# Autodesk Inventor assembly: Rebuild Chassis Assembly 26x28 Version with Shooter Tower
(part 2 of 2)
- Insert:77: Rebuild Shooter Tower Motor Mount Tube:1 ↔ 0.25x20 Washer:38
- Insert:78: Rebuild Shooter Tower Motor Mount Tube:1 ↔ 0.25x20 Washer:37
- Insert:79: Rebuild Snowblower Motor Mount:1 ↔ 0.25x20 Washer:39
- Insert:80: Rebuild Snowblower Motor Mount:1 ↔ 0.25x20 Washer:40
- Insert:81: Rebuild Snowblower Motor Mount:1 ↔ 0.25x20 Washer:41
- Insert:82: Rebuild Snowblower Motor Mount:1 ↔ 0.25x20 Washer:42
- Insert:83: Rebuild Shooter Tower Top Tube 1:1 ↔ 0.25x20 Washer:43
- Insert:84: Rebuild Shooter Tower Top Tube 1:1 ↔ 0.25x20 Washer:44
- Insert:85: 91257A548:1 ↔ 0.25x20 Washer:41
- Insert:86: 91257A548:2 ↔ 0.25x20 Washer:42
- Insert:87: 91257A548:3 ↔ 0.25x20 Washer:37
- Insert:88: 91257A548:4 ↔ 0.25x20 Washer:38
- Insert:89: 90630A110:22 ↔ 0.25x20 Washer:43
- Insert:90: 90630A110:21 ↔ 0.25x20 Washer:44
- Insert:91: 90630A110:24 ↔ 0.25x20 Washer:39
- Insert:92: 90630A110:23 ↔ 0.25x20 Washer:40
- Mate:324: Rebuild Shooter Tower Top Tube 1:1 ↔ Rebuild Flange Bearing Mount Tower:1
- Mate:325: Square Tube 3:1 ↔ Rebuild Flange Bearing Mount Tower Mirror:1
- Mate:326: Rebuild Shooter Tower Top Tube 1:1 ↔ Rebuild Flange Bearing Mount Tower:1
- Mate:327: Rebuild Shooter Tower Top Tube 1:1 ↔ Rebuild Flange Bearing Mount Tower:1
- Mate:328: Square Tube 3:1 ↔ Rebuild Flange Bearing Mount Tower Mirror:1
- Mate:329: Square Tube 3:1 ↔ Rebuild Flange Bearing Mount Tower Mirror:1
- Insert:93: Rebuild Gusset 4:3 ↔ 0.25x20 Washer:45
- Insert:94: Rebuild Gusset 4:3 ↔ 0.25x20 Washer:46
- Insert:95: Rebuild Gusset 4:5 ↔ 0.25x20 Washer:48
- Insert:96: Rebuild Gusset 4:5 ↔ 0.25x20 Washer:47
- Insert:97: 0.25x20 Washer:82 ↔ 91257A550:23
- Insert:98: 0.25x20 Washer:83 ↔ 91257A550:24
- Insert:99: Rebuild Flange Bearing Mount Tower Mirror:1 ↔ 91257A550:21
- Insert:100: Rebuild Flange Bearing Mount Tower Mirror:1 ↔ 91257A550:22
- Insert:101: 90630A110:26 ↔ 0.25x20 Washer:45
- Insert:102: 90630A110:25 ↔ 0.25x20 Washer:46
- Insert:103: 90630A110:27 ↔ 0.25x20 Washer:47
- Insert:104: 90630A110:28 ↔ 0.25x20 Washer:48
- Insert:105: Chassis Tower Bracket Part2:2 ↔ 0.25x20 Washer:49
- Insert:106: 0.25x20 Washer:50 ↔ Chassis Battery Mount Part1:1
- Insert:107: 0.25x20 Washer:50 ↔ 91257A548:5
- Insert:108: 0.25x20 Washer:49 ↔ 90630A110:29
- Insert:109: Chassis Tower Bracket Part2:1 ↔ 0.25x20 Washer:51
- Insert:110: 0.25x20 Washer:52 ↔ Chassis Battery Mount Part1:1
- Insert:111: 0.25x20 Washer:52 ↔ 91257A548:6
- Insert:112: 0.25x20 Washer:51 ↔ 90630A110:30
- Insert:113: Chassis Back Electronics Protector Bar:1 ↔ 0.25x20 Washer:53
- Insert:114: 0.25x20 Washer:54 ↔ Rebuild Mounting Board 3:1
- Insert:115: 0.25x20 Washer:53 ↔ 90630A110:31
- Insert:116: 0.25x20 Washer:54 ↔ 91257A548:7
- Mate:330: Chassis Part4 (26x28):1 ↔ Mounting Bracket V1.500 - (toughbox-mini - sheet metal - underside):2
- Mate:331: Chassis Part4 (26x28):1 ↔ Mounting Bracket V1.500 - (toughbox-mini - sheet metal):1
- Mate:332: Chassis Part4 (26x28):2 ↔ Mounting Bracket V1.500 - (toughbox-mini - sheet metal - underside):1
- Mate:333: Chassis Part4 (26x28):2 ↔ Mounting Bracket V1.500 - (toughbox-mini - sheet metal):2
- Mate:334: Chassis Part4 (26x28):2 ↔ Mounting Bracket V1.500 - (toughbox-mini - sheet metal):2
- Mate:335: Chassis Part4 (26x28):2 ↔ Mounting Bracket V1.500 - (toughbox-mini - sheet metal):2
- Mate:336: Chassis Part4 (26x28):1 ↔ Mounting Bracket V1.500 - (toughbox-mini - sheet metal):1
- Mate:337: Chassis Part4 (26x28):1 ↔ Mounting Bracket V1.500 - (toughbox-mini - sheet metal):1
- Mate:338: Chassis Part4 (26x28):1 ↔ Mounting Bracket V1.500 - (toughbox-mini - sheet metal - underside):2
- Mate:339: Chassis Part4 (26x28):1 ↔ Mounting Bracket V1.500 - (toughbox-mini - sheet metal - underside):2
- Mate:340: Chassis Part4 (26x28):2 ↔ Mounting Bracket V1.500 - (toughbox-mini - sheet metal - underside):1
- Mate:341: Chassis Part4 (26x28):2 ↔ Mounting Bracket V1.500 - (toughbox-mini - sheet metal - underside):1
- Insert:117: 0.25x20 Washer:56 ↔ Mounting Bracket V1.500 - (toughbox-mini - sheet metal):2
- Insert:118: 0.25x20 Washer:55 ↔ Mounting Bracket V1.500 - (toughbox-mini - sheet metal):2
- Insert:119: 0.25x20 Washer:57 ↔ Mounting Bracket V1.500 - (toughbox-mini - sheet metal):1
- Insert:120: 0.25x20 Washer:58 ↔ Mounting Bracket V1.500 - (toughbox-mini - sheet metal):1
- Insert:121: 0.25x20 Washer:60 ↔ Mounting Bracket V1.500 - (toughbox-mini - sheet metal - underside):1
- Insert:122: 0.25x20 Washer:59 ↔ Mounting Bracket V1.500 - (toughbox-mini - sheet metal - underside):1
- Insert:123: 0.25x20 Washer:61 ↔ Mounting Bracket V1.500 - (toughbox-mini - sheet metal - underside):2
- Insert:124: 0.25x20 Washer:62 ↔ Mounting Bracket V1.500 - (toughbox-mini - sheet metal - underside):2
- Insert:125: 91257A550:25 ↔ 0.25x20 Washer:56
- Insert:126: 91257A550:26 ↔ 0.25x20 Washer:55
- Insert:127: 91257A550:27 ↔ 0.25x20 Washer:57
- Insert:128: 91257A550:28 ↔ 0.25x20 Washer:58
- Insert:129: 90630A110:32 ↔ 0.25x20 Washer:60
- Insert:130: 90630A110:33 ↔ 0.25x20 Washer:59
- Insert:131: 90630A110:34 ↔ 0.25x20 Washer:62
- Insert:132: 90630A110:35 ↔ 0.25x20 Washer:61
- Mate:342: Rebuild Edge Mount 1:2 ↔ Back Brace Mount V2:1
- Flush:75: Rebuild Edge Mount 1:2 ↔ Back Brace Mount V2:1
- Mate:343 (155.2575 mm): Chassis V1.500 Part2:1 ↔ Back Brace Mount V2:1
- Mate:344: Circuit Breaker Mount:1 ↔ Back Brace Mount V2:1
- Mate:345: Circuit Breaker Mount:1 ↔ Back Brace Mount V2:1
- Mate:346: Circuit Breaker Mount:1 ↔ Back Brace Mount V2:1
- Insert:133: Rebuild Edge Mount 1:2 ↔ 0.25x20 Washer:65
- Insert:135: Rebuild Edge Mount 1:2 ↔ 0.25x20 Washer:63
- Insert:136: 0.25x20 Washer:66 ↔ Back Brace Mount V2:1
- Insert:138: 0.25x20 Washer:68 ↔ Back Brace Mount V2:1
- Insert:139: 0.25x20 Washer:69 ↔ Back Brace Mount V2:1
- Insert:140: 0.25x20 Washer:70 ↔ Back Brace Mount V2:1
- Insert:141: 0.25x20 Washer:71 ↔ Circuit Breaker Mount:1
- Insert:142: 0.25x20 Washer:72 ↔ Circuit Breaker Mount:1
- Insert:143: 91257A548:8 ↔ 0.25x20 Washer:66
- Insert:145: 91257A548:10 ↔ 0.25x20 Washer:68
- Insert:146: 90630A110:38 ↔ 0.25x20 Washer:63
- Insert:148: 90630A110:36 ↔ 0.25x20 Washer:65
- Insert:149: 92620A540:2 ↔ 0.25x20 Washer:71
- Insert:150: 92620A540:1 ↔ 0.25x20 Washer:72
- Insert:151: 90630A110:40 ↔ 0.25x20 Washer:69
- Insert:152: 90630A110:39 ↔ 0.25x20 Washer:70
- Flush:76 (0.7937 mm): Rebuild Shooter Tower Top Tube 1:1 ↔ Rebuild Snowblower Motor Mount:1
- Insert:155: Rebuild Gusset 4:4 ↔ 0.25x20 Washer:76
- Insert:156: Rebuild Gusset 4:4 ↔ 0.25x20 Washer:75
- Insert:157: 0.25x20 Washer:74 ↔ 91257A548:11
- Insert:158: 0.25x20 Washer:73 ↔ 91257A548:12
- Insert:159: 0.25x20 Washer:76 ↔ 90630A110:42
- Insert:160: 0.25x20 Washer:75 ↔ 90630A110:41
- Mate:350: Rebuild Encoder Mount 2:1 ↔ Rebuild Snowblower Motor Mount:1
- Mate:351: Rebuild Encoder Mount 2:1 ↔ Rebuild Snowblower Motor Mount:1
- Mate:352: Rebuild Encoder Mount 2:1 ↔ Rebuild Snowblower Motor Mount:1
- Insert:161: 90630A110:43 ↔ 0.25x20 Washer:79
- Insert:162: Rebuild Snowblower Motor Mount:1 ↔ 0.25x20 Washer:77
- Insert:163: 0.25x20 Washer:77 ↔ 92620A540:3
- Insert:164: Rebuild Encoder Mount 2:1 ↔ 0.25x20 Washer:78
- Insert:165: Rebuild Encoder Mount 2:1 ↔ 0.25x20 Washer:79
- Insert:166: 90630A110:44 ↔ 0.25x20 Washer:78
- Insert:167: Rebuild Snowblower Motor Mount:1 ↔ 92620A539:1
- Insert:168: Chassis V1.500 Part2:1 ↔ 0.25x20 Washer:80
- Insert:169: 0.25x20 Washer:80 ↔ 90630A110:45
- Insert:170: 0.25x20 Washer:81 ↔ Rebuild Mounting Board 3:1
- Insert:171: 0.25x20 Washer:81 ↔ 91257A548:13
- Insert:172: Rebuild Flange Bearing Mount Tower:1 ↔ 0.25x20 Washer:82
- Insert:173: Rebuild Flange Bearing Mount Tower:1 ↔ 0.25x20 Washer:83
- Insert:174: 0.25x20 Washer:84 ↔ 0.25x20 Washer:85
- Insert:175: 0.25x20 Washer:86 ↔ 0.25x20 Washer:85
- Insert:176: 0.25x20 Washer:86 ↔ 0.25x20 Washer:87
- Insert:177: 0.25x20 Washer:87 ↔ 0.25x20 Washer:88
- [Insert]: 0.25x20 Washer:89 ↔ 0.25x20 Washer:90
- [Insert]: 0.25x20 Washer:91 ↔ 0.25x20 Washer:90
- Insert:180: 0.25x20 Washer:88 ↔ 0.25x20 Washer:89
- [Insert]: 0.25x20 Washer:92 ↔ 0.25x20 Washer:93
- [Insert]: 0.25x20 Washer:94 ↔ 0.25x20 Washer:93
- [Insert]: 0.25x20 Washer:94 ↔ 0.25x20 Washer:95
- [Insert]: 0.25x20 Washer:96 ↔ 0.25x20 Washer:95
- [Insert]: 0.25x20 Washer:98 ↔ 0.25x20 Washer:97
- [Insert]: 0.25x20 Washer:99 ↔ 0.25x20 Washer:98
- [Insert]: 0.25x20 Washer:97 ↔ 0.25x20 Washer:96
- Insert:188: Rebuild Snowblower Motor Mount:1 ↔ 0.25x20 Washer:84
- Insert:189: Rebuild Snowblower Motor Mount:1 ↔ 0.25x20 Washer:92
- Angle:1 (0 deg): Rebuild Shooter Tower Motor Mount Tube:1 ↔ 92620A539:1
- Insert:190: Chassis V1.500 Part2:1 ↔ Chassis Back Electronics Protector Bar:1
- Flush:77: Chassis V1.500 Part2:1 ↔ Chassis Back Electronics Protector Bar:1
- Insert:191: Chassis Back Electronics Protector Bar:1 ↔ 0.25x20 Washer:100
- Insert:192: 90630A110:46 ↔ 0.25x20 Washer:100
- Insert:193: 0.25x20 Washer:101 ↔ Rebuild Shooter Tower Top Tube 2:1
- Insert:194: 0.25x20 Washer:101 ↔ 91257A548:14
- Mate:353: Limit Switch Bracket Shooter Front Right Corner:1 ↔ Rebuild Shooter Tower Top Tube 1:1
- Mate:354: Limit Switch Bracket Shooter Front Right Corner:1 ↔ Rebuild Shooter Tower Top Tube 1:1
- Mate:355: Limit Switch Bracket Shooter Front Right Corner:1 ↔ Rebuild Shooter Tower Top Tube 1:1
- Insert:195: Limit Switch Bracket Shooter Front Right Corner:1 ↔ 0.25x20 Washer:73
- Insert:196: Limit Switch Bracket Shooter Front Right Corner:1 ↔ 0.25x20 Washer:74
- Insert:197: 0.25x20 Washer:102 ↔ 0.25x20 Washer:91
- Insert:198: 0.25x20 Washer:103 ↔ 0.25x20 Washer:99
- Mate:356: Shooter Main Gear Guide Bar:1 ↔ 0.25x20 Washer:104
- Mate:357: Shooter Main Gear Guide Bar:1 ↔ Rebuild Snowblower Motor Mount:1
- Mate:358: Shooter Main Gear Guide Bar:1 ↔ Rebuild Snowblower Motor Mount:1
- Insert:199: 0.25x20 Washer:102 ↔ 0.25x20 Washer:104
- Insert:200: 0.25x20 Washer:103 ↔ 0.25x20 Washer:105
- Insert:201: Shooter Main Gear Guide Bar:1 ↔ 90630A110:47
- Insert:202: Shooter Main Gear Guide Bar:1 ↔ 90630A110:48
- Insert:203: 92620A542:2 ↔ Rebuild Snowblower Motor Mount:1
- Insert:204: 92620A542:1 ↔ Rebuild Snowblower Motor Mount:1
- Insert:205: 0.25x20 Washer Large Diameter:1 ↔ Chassis Part4 (26x28):2
- Insert:206: 0.25x20 Washer Large Diameter:1 ↔ 0.25x20 Washer Large Diameter:2
- Insert:207: 0.25x20 Washer Large Diameter:2 ↔ 0.25x20 Washer Large Diameter:3
- Insert:208: 0.25x20 Washer Large Diameter:3 ↔ 0.25x20 Washer Large Diameter:4
- Insert:209: 0.25x20 Washer Large Diameter:5 ↔ Chassis Part9 (26x28):2
- Insert:210: 0.25x20 Washer Large Diameter:5 ↔ 0.25x20 Washer Large Diameter:6
- Insert:211: 0.25x20 Washer Large Diameter:6 ↔ 0.25x20 Washer Large Diameter:7
- Insert:212: 0.25x20 Washer Large Diameter:7 ↔ 0.25x20 Washer Large Diameter:8
- Mate:359: 0.25x20 Washer Large Diameter:8 ↔ Chassis_Channel_AndyMark (4.5 inch):1
- Mate:360: 0.25x20 Washer Large Diameter:8 ↔ Chassis_Channel_AndyMark (4.5 inch):1
- [Insert]: 0.25x20 Washer:106 ↔ 90630A110:49
- Insert:214: Chassis_Channel_AndyMark (4.5 inch):1 ↔ 0.25x20 Washer:106
- Angle:2 (-73 deg): Chassis_Channel_AndyMark (4.5 inch):1 ↔ Chassis Part4 (26x28):2
- Mate:361: Chassis_Channel_AndyMark (4.5 inch):1 ↔ Chassis Part4 (26x28):2
- [Insert]: 0.25x20 Washer:107 ↔ 90630A110:50
- Insert:216: Chassis_Channel_AndyMark (4.5 inch):1 ↔ 0.25x20 Washer:107
- Insert:217 (31.75 mm): 3014T902:1 ↔ Chassis Part1 (26x28):1
- Insert:218 (31.75 mm): 3014T902:2 ↔ Chassis Part1 (26x28):2
- Mate:362: 3014T902:1 ↔ 3014T902:2
- Insert:219: 0.25x20 Washer:108 ↔ Chassis Part1 (26x28):1
- Insert:220: 0.25x20 Washer:109 ↔ Chassis Part1 (26x28):2
- Insert:221: 0.25x20 Washer:108 ↔ 90630A110:51
- Insert:222: 0.25x20 Washer:109 ↔ 90630A110:52
- [Insert]: 0.25x20 Washer:110 ↔ 90630A110:53
- Insert:224: 0.25x20 Washer:110 ↔ Chassis Part1 (26x28):1
- [Insert]: 0.25x20 Washer:111 ↔ 90630A110:54
- Insert:226: 0.25x20 Washer:111 ↔ Chassis Part1 (26x28):2
- Insert:227: 0.25x20 Washer:112 ↔ Chassis Part9 (26x28):2
- Insert:228: 0.25x20 Washer:113 ↔ Chassis Part4 (26x28):2
- Insert:229: 0.25x20 Washer:113 ↔ 91257A550:29
- Insert:230: 0.25x20 Washer:112 ↔ 91257A550:30
## Named parameters: d639_d637 = 0 mm, d640_d638 = 0 mm, d642_d641 = 0 mm, d643_d635 = 0 mm, d644_d636 = 0 mm, d645_d637 = 0 mm, d646_d638 = 0 mm, d647_d639_d637 = 0 mm, d648_d640_d638 = 0 mm, d684_d493 = 0 mm, d688_d684_d493 = 0 mm, d697_d498 = 0 mm, d699_d498 = 0 mm
